# Autodesk Inventor assembly: Ring B Assembly
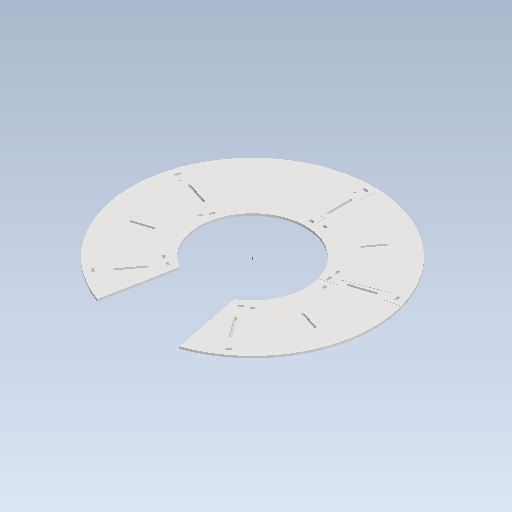
[picture p0: Inventor's stored thumbnail of the model, 512x512]
Saved by Autodesk Inventor 2020 (Build 240168000, 168)
## iProperties
Created: 2020-03-11
Part Number: Ring B Assembly
Document SubType Name: Assembly
Designer: danny
Author: danny
## Documents named in this file (5)
- C:\Users\Dan Wikman\OneDrive\University Life\2020, Semester 1\METR4900 Honours Thesis\Prototype CAD\Ring B Assembly.iam
- C:\Users\Dan Wikman\OneDrive\University Life\2020, Semester 1\METR4900 Honours Thesis\Prototype CAD\Ring B1.ipt
- C:\Users\Dan Wikman\OneDrive\University Life\2020, Semester 1\METR4900 Honours Thesis\Prototype CAD\Ring B2.ipt
- C:\Users\Dan Wikman\OneDrive\University Life\2020, Semester 1\METR4900 Honours Thesis\Prototype CAD\Ring B3.ipt
- C:\Users\Dan Wikman\OneDrive\University Life\2020, Semester 1\METR4900 Honours Thesis\Prototype CAD\Ring B4.ipt
## Components (4 placed, 4 different names)
1. Ring B1:1 — Flush:1, Mate:5, Mate:6
2. Ring B2:1 — Flush:1, Flush:2, Mate:1, Mate:2, Mate:5, Mate:6
3. Ring B3:1 — Flush:2, Flush:3, Mate:1, Mate:2, Mate:3, Mate:4
4. Ring B4:1 — Flush:3, Mate:3, Mate:4
## Relationships (9: Mate 6, Flush 3)
- Flush:1: Ring B1:1 ↔ Ring B2:1
- Flush:2: Ring B2:1 ↔ Ring B3:1
- Flush:3: Ring B3:1 ↔ Ring B4:1
- Mate:1: Ring B2:1 ↔ Ring B3:1
- Mate:2: Ring B2:1 ↔ Ring B3:1
- Mate:3: Ring B3:1 ↔ Ring B4:1
- Mate:4: Ring B3:1 ↔ Ring B4:1
- Mate:5: Ring B1:1 ↔ Ring B2:1
- Mate:6: Ring B1:1 ↔ Ring B2:1
